# Autodesk Inventor assembly: mirror mount
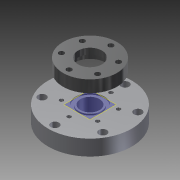
[picture p0: Inventor's stored thumbnail of the model, 180x180]
Saved by Autodesk Inventor 2014 (Build 180170000, 170)
## iProperties
Created: 2011-05-26
Part Number: mirror mount
Document SubType Name: Assembly
Designer: ijs09
Author: ijs09
## Documents named in this file (3)
- D:\Inventor\Aki Pump Window Mount\mirror mount.iam
- D:\Inventor\Aki Pump Window Mount\Conflat Flange.ipt
- D:\Inventor\Aki Pump Window Mount\nylon clamp.ipt
## Components (2 placed, 2 different names)
1. Conflat Flange:1 — Mate:1, Mate:2
2. nylon clamp:1 — Mate:1, Mate:2
## Relationships (2: Mate 2)
- Mate:1: Conflat Flange:1 ↔ nylon clamp:1
- Mate:2: Conflat Flange:1 ↔ nylon clamp:1
